# Autodesk Inventor assembly: A2017_T5_04
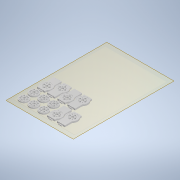
[picture p0: Inventor's stored thumbnail of the model, 180x180]
Saved by Autodesk Inventor 2020 (Build 240168000, 168)
## iProperties
Created: 2021-08-27
Part Number: A2017_T5_04
Document SubType Name: Assembly
Designer: Masato
Author: Masato
## Documents named in this file (4)
- C:\Inventor\SUSTAINA-OP\Cam\A2017_T5_04.iam
- C:\Inventor\SUSTAINA-OP\Cam\DisposableBoard.ipt
- C:\Inventor\SUSTAINA-OP\UpperBody\Trunk\CrossRollerBearing\Inner_support_stand.ipt
- C:\Inventor\SUSTAINA-OP\LowerBody\Leg_joint\Leg_joint_yaw_frame.ipt
## Components (13 placed, 3 different names)
1. DisposableBoard:1 — メイト:2, メイト:1, フラッシュ:1, フラッシュ:2, メイト:20, 角度:4, 正接:1, 正接:2, メイト:21, メイト:22, メイト:23, メイト:24, フラッシュ:3, 正接:6, 角度:5
2. Leg_joint_yaw_frame:1 — メイト:21, フラッシュ:3, 正接:3, フラッシュ:4, 正接:4
3. Leg_joint_yaw_frame:3 — メイト:22, フラッシュ:4, 正接:4
4. Inner_support_stand:1 — メイト:20, 角度:4, 正接:1, 正接:2
5. Inner_support_stand:2
6. Inner_support_stand:3 — 正接:3
7. Inner_support_stand:4 — 正接:5
8. Inner_support_stand:5
9. Inner_support_stand:6
10. Leg_joint_yaw_frame:2 — メイト:23, 正接:5, 正接:6, 角度:5, フラッシュ:5, 正接:7
11. Leg_joint_yaw_frame:4 — メイト:24, フラッシュ:5, 正接:7
12. Leg_joint_yaw_frame:5
13. Leg_joint_yaw_frame:6
## Component patterns: (6 elements, first: Inner_support_stand:1), (2 elements, first: Leg_joint_yaw_frame:2 + Leg_joint_yaw_frame:4)
## Relationships (21: Mate 7, Tangent 7, Flush 5, Angle 2)
- メイト:2 [Mate]: DisposableBoard:1
- メイト:1 [Mate]: DisposableBoard:1
- フラッシュ:1 [Flush]: DisposableBoard:1
- フラッシュ:2 [Flush]: DisposableBoard:1
- メイト:20 [Mate]: DisposableBoard:1 ↔ Inner_support_stand:1
- 角度:4 [Angle] (0 deg): DisposableBoard:1 ↔ Inner_support_stand:1
- 正接:1 [Tangent] (2 mm): DisposableBoard:1 ↔ Inner_support_stand:1
- 正接:2 [Tangent] (2 mm): DisposableBoard:1 ↔ Inner_support_stand:1
- メイト:21 [Mate]: DisposableBoard:1 ↔ Leg_joint_yaw_frame:1
- メイト:22 [Mate]: DisposableBoard:1 ↔ Leg_joint_yaw_frame:3
- メイト:23 [Mate]: DisposableBoard:1 ↔ Leg_joint_yaw_frame:2
- メイト:24 [Mate]: DisposableBoard:1 ↔ Leg_joint_yaw_frame:4
- フラッシュ:3 [Flush] (2 mm): DisposableBoard:1 ↔ Leg_joint_yaw_frame:1
- 正接:3 [Tangent] (3.5 mm): Leg_joint_yaw_frame:1 ↔ Inner_support_stand:3
- フラッシュ:4 [Flush]: Leg_joint_yaw_frame:1 ↔ Leg_joint_yaw_frame:3
- 正接:4 [Tangent] (2.5 mm): Leg_joint_yaw_frame:1 ↔ Leg_joint_yaw_frame:3
- 正接:5 [Tangent] (2.5 mm): Inner_support_stand:4 ↔ Leg_joint_yaw_frame:2
- 正接:6 [Tangent] (2 mm): DisposableBoard:1 ↔ Leg_joint_yaw_frame:2
- 角度:5 [Angle] (0 deg): DisposableBoard:1 ↔ Leg_joint_yaw_frame:2
- フラッシュ:5 [Flush]: Leg_joint_yaw_frame:2 ↔ Leg_joint_yaw_frame:4
- 正接:7 [Tangent] (2.5 mm): Leg_joint_yaw_frame:2 ↔ Leg_joint_yaw_frame:4
